# Autodesk Inventor assembly: 4.1h_JulianR_Assemblypart2
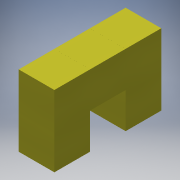
[picture p0: Inventor's stored thumbnail of the model, 180x180]
Saved by Autodesk Inventor 2016 (Build 200138000, 138)
## iProperties
Created: 2017-03-02
Part Number: 4.1h_JulianR_Assemblypart2
Document SubType Name: Assembly
Designer: fhs-mgr
Author: fhs-mgr
## Documents named in this file (2)
- H:\IED 5th Inventor\4.1h_JulianR_Assemblypart2.iam
- H:\IED 5th Inventor\WoodenBlock.ipt
## Components (5 placed, 1 different names)
1. WoodenBlock:1 — Mate:1, Mate:2, Mate:3, Mate:4, Mate:8
2. WoodenBlock:2 — Mate:1, Mate:2, Mate:7
3. WoodenBlock:3 — Mate:3, Mate:4, Mate:5, Mate:6
4. WoodenBlock:4 — Mate:5, Mate:6
5. WoodenBlock:5 — Mate:7, Mate:8
## Relationships (8: Mate 8)
- Mate:1: WoodenBlock:1 ↔ WoodenBlock:2
- Mate:2: WoodenBlock:1 ↔ WoodenBlock:2
- Mate:3: WoodenBlock:1 ↔ WoodenBlock:3
- Mate:4: WoodenBlock:1 ↔ WoodenBlock:3
- Mate:5: WoodenBlock:3 ↔ WoodenBlock:4
- Mate:6: WoodenBlock:3 ↔ WoodenBlock:4
- Mate:7: WoodenBlock:2 ↔ WoodenBlock:5
- Mate:8: WoodenBlock:1 ↔ WoodenBlock:5
